# Autodesk Inventor assembly: 400mm_X95_with_base_and_clamp
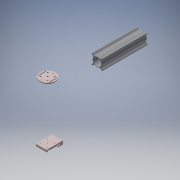
[picture p0: Inventor's stored thumbnail of the model, 180x180]
Saved by Autodesk Inventor 2016 (Build 200138000, 138)
## iProperties
Created: 2018-09-27
Part Number: 400mm_X95_with_base_and_clamp
Document SubType Name: Assembly
Designer: voigt
Author: voigt
## Documents named in this file (4)
- D:\Microscope_Design\CAD_Files\mesoSPIM_design\mesoSPIM\sample_stages\400mm_X95_with_base_and_clamp.iam
- D:\Microscope_Design\CAD_Files\mesoSPIM_design\library\Qioptiq\X95_accessoires\X95_baseplate.ipt
- D:\Microscope_Design\CAD_Files\mesoSPIM_design\library\Qioptiq\X95_carriers\X95_clamping_carrier.ipt
- D:\Microscope_Design\CAD_Files\mesoSPIM_design\library\Qioptiq\X95_rails\X95_400mm.ipt
## Components (3 placed, 3 different names)
1. X95_baseplate:1
2. X95_400mm:1
3. X95_clamping_carrier:1
## Relationships (6: Mate 6)
- [Mate]: X95_baseplate:1 ↔ X95_400mm:1
- [Mate]: X95_baseplate:1 ↔ X95_400mm:1
- [Mate]: X95_baseplate:1 ↔ X95_400mm:1
- [Mate]: X95_400mm:1 ↔ X95_clamping_carrier:1
- [Mate]: X95_400mm:1 ↔ X95_clamping_carrier:1
- [Mate]: X95_400mm:1 ↔ X95_clamping_carrier:1
